# Autodesk Inventor assembly: bellows_latest
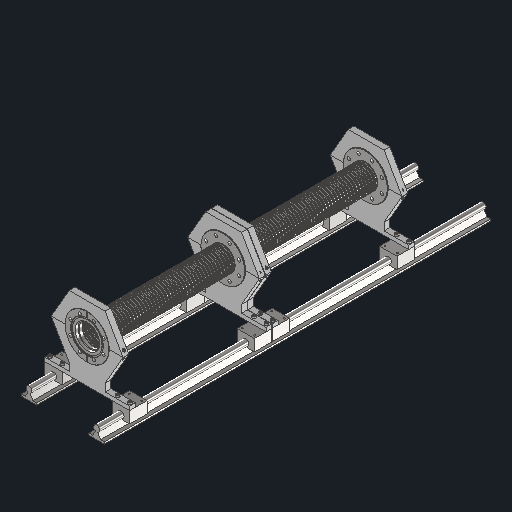
[picture p0: Inventor's stored thumbnail of the model, 512x512]
Saved by Autodesk Inventor 2027.1 (Build 311270010, 270A)
## iProperties
Created: 2026-06-04
Part Number: bellows_latest
Document SubType Name: Assembly
Designer: shusu
Author: shusu
## Documents named in this file (3)
- C:\Users\queezz\Dropbox\Drawings\PIHTI\bellows\bellows.iam
- C:\Users\queezz\Dropbox\Drawings\PIHTI\bellows\rail.ipt
- C:\Users\queezz\Dropbox\Drawings\PIHTI\bellows\bellows_2.iam
## Components (4 placed, 2 different names)
1. rail:1 — Insert:2
2. rail:2 — Insert:1
3. bellows_2:1 [sub-assembly] — Insert:1, Insert:2, Mate:1
4. bellows_2:2 [sub-assembly] — Mate:1
## Relationships (3: Insert 2, Mate 1)
- Insert:1 (-800 mm): rail:2 ↔ bellows_2:1
- Insert:2 (-800 mm): rail:1 ↔ bellows_2:1
- Mate:1: bellows_2:1 ↔ bellows_2:2
